# Autodesk Inventor assembly: Camera with Clip
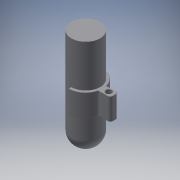
[picture p0: Inventor's stored thumbnail of the model, 180x180]
Saved by Autodesk Inventor 2019.4 (Build 234330000, 330)
## iProperties
Created: 2021-02-04
Part Number: Camera with Clip
Document SubType Name: Assembly
Designer: caleb
Author: caleb
## Documents named in this file (3)
- C:\Users\cfang\Desktop\nebraska-silicon-lab\CAD\Pull Tester\Camera with Clip.iam
- C:\Users\cfang\Desktop\nebraska-silicon-lab\CAD\Pull Tester\Camera Clip.ipt
- C:\Users\cfang\Desktop\nebraska-silicon-lab\CAD\Pull Tester\Camera.ipt
## Components (2 placed, 2 different names)
1. Camera Clip:1 — Mate:1
2. Camera:1 — Mate:1
## Relationships (1: Mate 1)
- Mate:1: Camera Clip:1 ↔ Camera:1
